# Autodesk Inventor assembly: 클램프
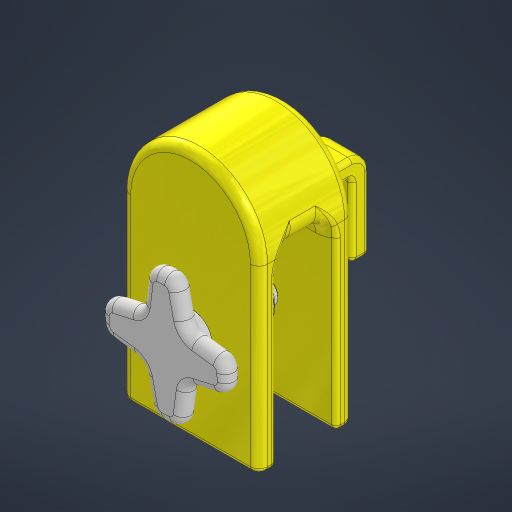
[picture p0: Inventor's stored thumbnail of the model, 512x512]
Saved by Autodesk Inventor 2024 (Build 280153000, 153)
## iProperties
Created: 2024-01-30
Part Number: 클램프
Document SubType Name: Assembly
Designer: KBU
Author: KBU
## Documents named in this file (3)
- D:\github\Modeling\IKEA 페그보드 시제품\클램프.iam
- D:\github\Modeling\IKEA 페그보드 시제품\부품1.ipt
- D:\github\Modeling\IKEA 페그보드 시제품\부품2.ipt
## Components (2 placed, 2 different names)
1. 부품1:1 — 삽입:1
2. 부품2:1 — 삽입:1
## Relationships (1: Insert 1)
- 삽입:1 [Insert] (-3 mm): 부품1:1 ↔ 부품2:1
